# Autodesk Inventor assembly: UBG-Dribblerhalter
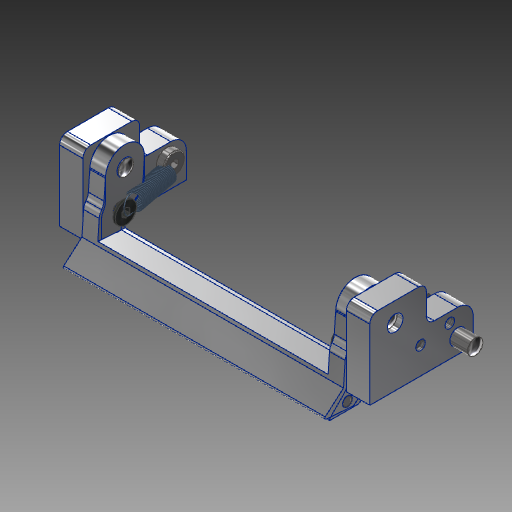
[picture p0: Inventor's stored thumbnail of the model, 512x512]
Saved by Autodesk Inventor 2019.4 (Build 234330000, 330)
## iProperties
Part Number: UBG-Dribblerhalter
Material: Generisch
Document SubType Name: Assembly
Designer: rYan
Mass: 41.0398 g
Surface Area: 116.754 cm^2
Volume: 13.2404 cm^3
Density: 3.09957 g/cm^3
Author: rYan
## Documents named in this file (8)
- D:\TIGERsGIT\Hardware\mechanik\2020\Inventor\Robot\Dribbler\UBG-Dribblerhalter.iam
- D:\TIGERsGIT\Hardware\mechanik\2020\Inventor\Robot\Dribbler\Dribbler Lagerbock.ipt
- D:\TIGERsGIT\Hardware\mechanik\2020\Inventor\Inhaltscenter\de-DE\ISO 8745(2)\ISO 8745 - 4 x 10(6).ipt
- D:\TIGERsGIT\Hardware\mechanik\2020\Inventor\Robot\Kicker\Chip Schaufel.ipt
- D:\TIGERsGIT\Hardware\mechanik\2020\Inventor\Purchased Parts\Zugfeder RZ-006DI.ipt
- D:\TIGERsGIT\Hardware\mechanik\2020\Inventor\Robot\Kicker\MG-Chip Schaufel.iam
- D:\TIGERsGIT\Hardware\mechanik\2020\Inventor\Inhaltscenter\de-DE\DIN 7984\DIN 7984 - M3 x 5.ipt
- D:\TIGERsGIT\Hardware\mechanik\2020\Inventor\Purchased Parts\ISO 10642 - M3 x  6.ipt
## Components (14 placed, 7 different names)
1. Dribbler Lagerbock:1 — Passend:2, Passend:4, Symmetrie:1, Passend:5, Einfügen:2, Einfügen:4, Passend:6, Winkel:1, Einfügen:5, Winkel:2
2. Dribbler Lagerbock:2 — Passend:1, Passend:3, Symmetrie:1, Passend:5, Einfügen:1, Einfügen:3, Passend:7, Einfügen:6, Einfügen:8
3. DIN EN ISO 8745 4 x 10:1 — Einfügen:1
4. DIN EN ISO 8745 4 x 10:2 — Einfügen:2
5. DIN EN ISO 8745 4 x 10:3 — Einfügen:4
6. DIN EN ISO 8745 4 x 10:4 — Einfügen:3
7. Chip Schaufel:1 — Passend:6, Fluchtend:1, Winkel:1, Einfügen:9, Einfügen:10
8. Zugfeder RZ-006DI:1
9. MG-Chip Schaufel:1 [sub-assembly] — Fluchtend:2, Passend:7, Winkel:2
10. DIN 7984 M3 x 5:1 — Einfügen:5
11. DIN 7984 M3 x 5:2 — Einfügen:6
12. DIN 7984 M3 x 5:4 — Einfügen:8
13. ISO 10642 M3 x  6:1 — Einfügen:10
14. ISO 10642 M3 x  6:2 — Einfügen:9
## Relationships (21: Insert 9, Mate 7, Flush 2, Angle 2, Symmetry 1)
- Passend:1 [Mate]: Dribbler Lagerbock:2
- Passend:2 [Mate]: Dribbler Lagerbock:1
- Passend:3 [Mate]: Dribbler Lagerbock:2
- Passend:4 [Mate]: Dribbler Lagerbock:1
- Symmetrie:1: Dribbler Lagerbock:1 ↔ Dribbler Lagerbock:2
- Passend:5 [Mate] (67.5 mm): Dribbler Lagerbock:1 ↔ Dribbler Lagerbock:2
- Einfügen:1 [Insert] (1.5 mm): Dribbler Lagerbock:2 ↔ DIN EN ISO 8745 4 x 10:1
- Einfügen:2 [Insert] (1.5 mm): Dribbler Lagerbock:1 ↔ DIN EN ISO 8745 4 x 10:2
- Einfügen:3 [Insert] (1.5 mm): Dribbler Lagerbock:2 ↔ DIN EN ISO 8745 4 x 10:4
- Einfügen:4 [Insert] (1.5 mm): Dribbler Lagerbock:1 ↔ DIN EN ISO 8745 4 x 10:3
- Passend:6 [Mate]: Dribbler Lagerbock:1 ↔ Chip Schaufel:1
- Fluchtend:1 [Flush]: Chip Schaufel:1
- Winkel:1 [Angle] (0 deg): Dribbler Lagerbock:1 ↔ Chip Schaufel:1
- Fluchtend:2 [Flush]: MG-Chip Schaufel:1
- Passend:7 [Mate]: Dribbler Lagerbock:2 ↔ MG-Chip Schaufel:1
- Einfügen:5 [Insert] (1 mm): Dribbler Lagerbock:1 ↔ DIN 7984 M3 x 5:1
- Einfügen:6 [Insert] (1 mm): Dribbler Lagerbock:2 ↔ DIN 7984 M3 x 5:2
- Einfügen:8 [Insert]: Dribbler Lagerbock:2 ↔ DIN 7984 M3 x 5:4
- Winkel:2 [Angle] (0 deg): Dribbler Lagerbock:1 ↔ MG-Chip Schaufel:1
- Einfügen:9 [Insert]: Chip Schaufel:1 ↔ ISO 10642 M3 x  6:2
- Einfügen:10 [Insert]: Chip Schaufel:1 ↔ ISO 10642 M3 x  6:1
